# Autodesk Inventor assembly: HIN-61 BISAGRA (P2 PUERTA)
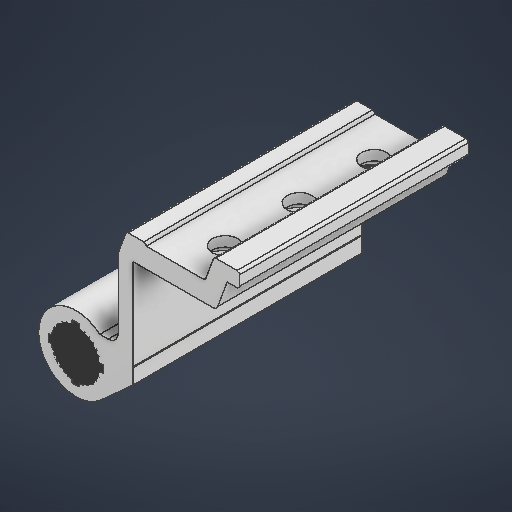
[picture p0: Inventor's stored thumbnail of the model, 512x512]
Saved by Autodesk Inventor 2025 (Build 290162000, 162)
## iProperties
Created: 2026-02-23
Part Number: HIN-61 BISAGRA (P2 PUERTA)
Document SubType Name: Assembly
Designer: ROLANDO
Author: ROLANDO
## Documents named in this file (4)
- C:\Users\rolan\OneDrive\Documentos\Inventor\Projects\CARPINTERIA ALUMINIO\PUERTAS Y VENTANAS\ACCESORIOS\BISAGRAS\ENSAMBLES\HIN-61 BISAGRA (P2 PUERTA).iam
- C:\Users\rolan\OneDrive\Documentos\Inventor\Projects\CARPINTERIA ALUMINIO\PUERTAS Y VENTANAS\ACCESORIOS\BISAGRAS\PIEZAS\HIN-61 BISAGRA\HIN-61 BISAGRA (P2 PUERTA).ipt
- C:\Users\rolan\OneDrive\Documentos\Inventor\Projects\CARPINTERIA ALUMINIO\PUERTAS Y VENTANAS\ACCESORIOS\BISAGRAS\PIEZAS\HIN-61 BISAGRA\HIN-61 BISAGRA (BUJE PLASTICO).ipt
- HIN-61 BISAGRA (P2 PUERTA).iam
## Components (2 placed, 2 different names)
1. HIN-61 BISAGRA (P2 PUERTA):1 — Coincidencia:1, Coincidencia:2, Coincidencia:3
2. HIN-61 BISAGRA (BUJE PLASTICO):1 — Coincidencia:1, Coincidencia:2, Coincidencia:3
## Relationships (3: Mate 3)
- Coincidencia:1 [Mate]: HIN-61 BISAGRA (P2 PUERTA):1 ↔ HIN-61 BISAGRA (BUJE PLASTICO):1
- Coincidencia:2 [Mate]: HIN-61 BISAGRA (P2 PUERTA):1 ↔ HIN-61 BISAGRA (BUJE PLASTICO):1
- Coincidencia:3 [Mate]: HIN-61 BISAGRA (P2 PUERTA):1 ↔ HIN-61 BISAGRA (BUJE PLASTICO):1
